# Autodesk Inventor assembly: DisplayModuleAssembly
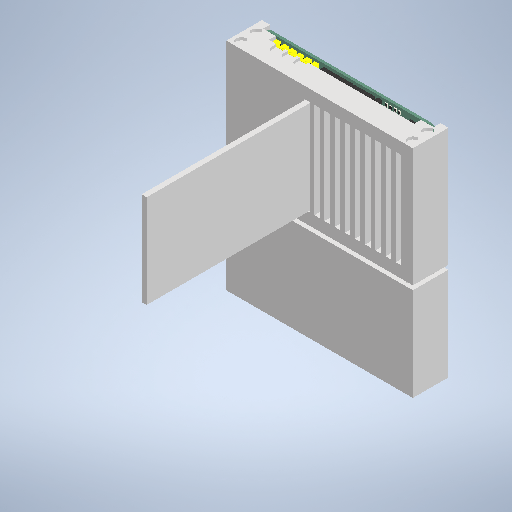
[picture p0: Inventor's stored thumbnail of the model, 512x512]
Saved by Autodesk Inventor 2025.1 (Build 291241020, 241B)
## iProperties
Created: 2024-09-25
Part Number: DisplayModuleAssembly
Document SubType Name: Assembly
Designer: Si Teng Wu
Author: Si Teng Wu
## Documents named in this file (7)
- C:\Users\Si Teng Wu\OneDrive - University of Cape Town\2024\EEE4022S\IOT_Retro_Display_EEE4022S\3D Models\DisplayModuleAssembly.iam
- C:\Users\Si Teng Wu\OneDrive - University of Cape Town\2024\EEE4022S\IOT_Retro_Display_EEE4022S\3D Models\DisplayModule.ipt
- C:\Users\Si Teng Wu\OneDrive - University of Cape Town\2024\EEE4022S\IOT_Retro_Display_EEE4022S\3D Models\DisplayModuleHousing.ipt
- C:\Users\Si Teng Wu\OneDrive - University of Cape Town\2024\EEE4022S\IOT_Retro_Display_EEE4022S\3D Models\AcrylicPane.ipt
- C:\Users\Si Teng Wu\OneDrive - University of Cape Town\2024\EEE4022S\IOT_Retro_Display_EEE4022S\3D Models\PowerModuleHousing.ipt
- C:\Users\Si Teng Wu\OneDrive - University of Cape Town\2024\EEE4022S\IOT_Retro_Display_EEE4022S\3D Models\DisplayModuleHousingCap.ipt
- C:\Users\Si Teng Wu\OneDrive - University of Cape Town\2024\EEE4022S\IOT_Retro_Display_EEE4022S\3D Models\PowerModule.ipt
## Components (6 placed, 6 different names)
1. DisplayModule:1 — Mate:6, Mate:7, Flush:1, Flush:4
2. DisplayModuleHousing:1 — Mate:6, Mate:7, Flush:1, Mate:8, Mate:9, Mate:10, Mate:11, Flush:2, Flush:3
3. AcrylicPane:1 — Mate:8, Mate:9, Mate:10, Mate:12, Mate:13, Mate:14
4. PowerModuleHousing:1 — Mate:11, Flush:2, Flush:3, Mate:16, Mate:17
5. DisplayModuleHousingCap:1 — Mate:12, Mate:13, Mate:14
6. PowerModule:1 — Flush:4, Mate:16, Mate:17
## Relationships (15: Mate 11, Flush 4)
- Mate:6 (0.25 mm): DisplayModule:1 ↔ DisplayModuleHousing:1
- Mate:7: DisplayModule:1 ↔ DisplayModuleHousing:1
- Flush:1: DisplayModule:1 ↔ DisplayModuleHousing:1
- Mate:8 (1 mm): DisplayModuleHousing:1 ↔ AcrylicPane:1
- Mate:9 (0.7 mm): DisplayModuleHousing:1 ↔ AcrylicPane:1
- Mate:10 (0.1 mm): DisplayModuleHousing:1 ↔ AcrylicPane:1
- Mate:11 (2.5 mm): DisplayModuleHousing:1 ↔ PowerModuleHousing:1
- Flush:2: DisplayModuleHousing:1 ↔ PowerModuleHousing:1
- Flush:3: DisplayModuleHousing:1 ↔ PowerModuleHousing:1
- Mate:12: AcrylicPane:1 ↔ DisplayModuleHousingCap:1
- Mate:13 (0.7 mm): AcrylicPane:1 ↔ DisplayModuleHousingCap:1
- Mate:14 (0.1 mm): AcrylicPane:1 ↔ DisplayModuleHousingCap:1
- Flush:4: DisplayModule:1 ↔ PowerModule:1
- Mate:16 (0.25 mm): PowerModuleHousing:1 ↔ PowerModule:1
- Mate:17: PowerModuleHousing:1 ↔ PowerModule:1
